# Autodesk Inventor assembly: Shooter Oct14
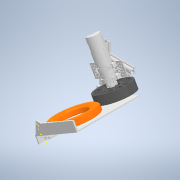
[picture p0: Inventor's stored thumbnail of the model, 180x180]
Saved by Autodesk Inventor 2020 (Build 240168000, 168)
## iProperties
Created: 2020-10-14
Part Number: Shooter Oct14
Document SubType Name: Assembly
Designer: Owner
Author: Owner
## Documents named in this file (11)
- C:\Users\tdmp4\Documents\GitHub\CAD-2021-Ultimate_Goal\Shooter\Shooter Oct14.iam
- C:\Users\tdmp4\Documents\GitHub\CAD-2021-Ultimate_Goal\ServoCity\7in-Xrail.ipt
- C:\Users\tdmp4\Documents\GitHub\CAD-2021-Ultimate_Goal\ServoCity\565018.ipt
- C:\Users\tdmp4\Documents\GitHub\CAD-2021-Ultimate_Goal\Shooter\Shooter plate but for an xrail.ipt
- C:\Users\tdmp4\Documents\GitHub\CAD-2021-Ultimate_Goal\ServoCity\585722.ipt
- C:\Users\tdmp4\Documents\GitHub\CAD-2021-Ultimate_Goal\GoBilda\5202-0002-0003 part.ipt
- C:\Users\tdmp4\Documents\GitHub\CAD-2021-Ultimate_Goal\ServoCity\555176 assembly.ipt
- C:\Users\tdmp4\Documents\GitHub\CAD-2021-Ultimate_Goal\AndyMark\am-3563 4IN 8mm Round Compliant Wheel REV2.ipt
- C:\Users\tdmp4\Documents\GitHub\CAD-2021-Ultimate_Goal\ServoCity\545456.ipt
- C:\Users\tdmp4\Documents\GitHub\CAD-2021-Ultimate_Goal\ServoCity\545636 assembly.ipt
- C:\Users\tdmp4\Documents\GitHub\CAD-2021-Ultimate_Goal\AndyMark\am-4300 Ring.ipt
## Components (12 placed, 10 different names)
1. 7in-Xrail:1 — Mate:1, Mate:2, Mate:4
2. 7in-Xrail:2 — Mate:3, Mate:4
3. 565018:1 — Mate:1, Mate:13
4. Shooter plate but for an xrail:1 — Mate:2, Mate:3, Mate:21
5. 585722:1 — Mate:5, Mate:6, Mate:7, Mate:8, Mate:11, Mate:12, Mate:13
6. 5202-0002-0003 part:1 — Mate:9, Mate:10, Mate:20, Mate:22
7. 555176 assembly:1 — Mate:5, Mate:8, Mate:9, Mate:12
8. 555176 assembly:2 — Mate:6, Mate:7, Mate:10, Mate:11
9. am-3563 4IN 8mm Round Compliant Wheel REV2:1 — Mate:19
10. 545456:1 — Mate:19
11. 545636 assembly:1 — Mate:20, Mate:22
12. am-4300 Ring:1 — Mate:21
## Relationships (22: Mate 22)
- Mate:1: 7in-Xrail:1 ↔ 565018:1
- Mate:2: 7in-Xrail:1 ↔ Shooter plate but for an xrail:1
- Mate:3: 7in-Xrail:2 ↔ Shooter plate but for an xrail:1
- Mate:4: 7in-Xrail:1 ↔ 7in-Xrail:2
- Mate:5: 585722:1 ↔ 555176 assembly:1
- Mate:6: 585722:1 ↔ 555176 assembly:2
- Mate:7: 585722:1 ↔ 555176 assembly:2
- Mate:8: 585722:1 ↔ 555176 assembly:1
- Mate:9: 5202-0002-0003 part:1 ↔ 555176 assembly:1
- Mate:10: 5202-0002-0003 part:1 ↔ 555176 assembly:2
- Mate:11: 585722:1 ↔ 555176 assembly:2
- Mate:12: 585722:1 ↔ 555176 assembly:1
- Mate:13: 565018:1 ↔ 585722:1
- [Mate]: 545456:1 ↔ 545636 assembly:1
- [Mate]: 545456:1 ↔ 545636 assembly:1
- [Mate]: 545456:1 ↔ 545636 assembly:1
- [Mate]: am-3563 4IN 8mm Round Compliant Wheel REV2:1 ↔ 545456:1
- [Mate]: am-3563 4IN 8mm Round Compliant Wheel REV2:1 ↔ 545456:1
- Mate:19: am-3563 4IN 8mm Round Compliant Wheel REV2:1 ↔ 545456:1
- Mate:20: 5202-0002-0003 part:1 ↔ 545636 assembly:1
- Mate:21: Shooter plate but for an xrail:1 ↔ am-4300 Ring:1
- Mate:22: 5202-0002-0003 part:1 ↔ 545636 assembly:1
## Named parameters: d13_d14 = 0 mm, d14_d17 = 0 mm
